# Autodesk Inventor assembly: FemaleHeaderPin_1x6
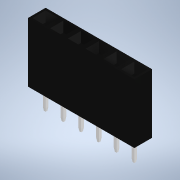
[picture p0: Inventor's stored thumbnail of the model, 180x180]
Saved by Autodesk Inventor 2021 (Build 250183000, 183)
## iProperties
Created: 2020-01-02
Part Number: FemaleHeaderPin_1x6
Document SubType Name: Assembly
Designer: ermoz
Author: ermoz
## Documents named in this file (2)
- D:\Moje Wyczyny\My_Poor_Projects\Sneak100_MiniSumo\minisumo-sneak100\mechanics\PreMadeParts\FemaleHeaderPin_1x6.iam
- D:\Moje Wyczyny\My_Poor_Projects\Sneak100_MiniSumo\minisumo-sneak100\mechanics\PreMadeParts\FemaleHederPin.ipt
## Components (6 placed, 1 different names)
1. FemaleHederPin:1 — Mate:1, Flush:1, Flush:7
2. FemaleHederPin:2 — Mate:1, Mate:2, Flush:1, Flush:2, Flush:7, Flush:8
3. FemaleHederPin:3 — Mate:2, Mate:3, Flush:2, Flush:3, Flush:8, Flush:9
4. FemaleHederPin:4 — Mate:3, Mate:4, Flush:3, Flush:4, Flush:9, Flush:10
5. FemaleHederPin:5 — Mate:4, Flush:4, Flush:10, Mate:5, Flush:11, Flush:12
6. FemaleHederPin:6 — Mate:5, Flush:11, Flush:12
## Relationships (15: Flush 10, Mate 5)
- Mate:1: FemaleHederPin:1 ↔ FemaleHederPin:2
- Mate:2: FemaleHederPin:2 ↔ FemaleHederPin:3
- Mate:3: FemaleHederPin:3 ↔ FemaleHederPin:4
- Mate:4: FemaleHederPin:4 ↔ FemaleHederPin:5
- Flush:1: FemaleHederPin:1 ↔ FemaleHederPin:2
- Flush:2: FemaleHederPin:2 ↔ FemaleHederPin:3
- Flush:3: FemaleHederPin:3 ↔ FemaleHederPin:4
- Flush:4: FemaleHederPin:4 ↔ FemaleHederPin:5
- Flush:7: FemaleHederPin:1 ↔ FemaleHederPin:2
- Flush:8: FemaleHederPin:2 ↔ FemaleHederPin:3
- Flush:9: FemaleHederPin:3 ↔ FemaleHederPin:4
- Flush:10: FemaleHederPin:4 ↔ FemaleHederPin:5
- Mate:5: FemaleHederPin:5 ↔ FemaleHederPin:6
- Flush:11: FemaleHederPin:5 ↔ FemaleHederPin:6
- Flush:12: FemaleHederPin:5 ↔ FemaleHederPin:6
